# Autodesk Inventor assembly: Neuronexus
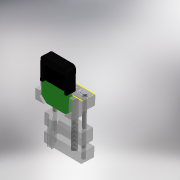
[picture p0: Inventor's stored thumbnail of the model, 180x180]
Saved by Autodesk Inventor 2020 (Build 240168000, 168)
## iProperties
Created: 2020-02-24
Part Number: Neuronexus
Document SubType Name: Assembly
Designer: Knowblesse
Author: Knowblesse
## Documents named in this file (7)
- C:\VCF\Microdrive\Neuronexus\Neuronexus.iam
- C:\VCF\Microdrive\Neuronexus\Bot.ipt
- C:\VCF\Microdrive\Neuronexus\Mid.ipt
- C:\VCF\Microdrive\Neuronexus\Screw.ipt
- C:\VCF\Microdrive\Neuronexus\Top.ipt
- C:\VCF\Microdrive\Neuronexus\19G_Pillar.ipt
- C:\VCF\Microdrive\Neuronexus\Probe.ipt
## Components (7 placed, 6 different names)
1. Bot:1 — 회전:4, 회전:5
2. Mid:1 — 원통형:2, 원통형:3
3. Screw:1 — 회전:1
4. Top:1 — 회전:1, 메이트:1, 회전:2, 회전:3, 강체:1
5. 19G_Pillar:1 — 메이트:1, 회전:3, 회전:4, 원통형:3
6. 19G_Pillar:2 — 원통형:2, 회전:2, 회전:5
7. Probe:1 — 강체:1
## Relationships (9: RevoluteJoint 5, CylindricalJoint 2, Mate 1, WeldJoint 1)
- 원통형:2 [CylindricalJoint]: Mid:1 ↔ 19G_Pillar:2
- 회전:1 [RevoluteJoint]: Screw:1 ↔ Top:1
- 메이트:1 [Mate]: Top:1 ↔ 19G_Pillar:1
- 회전:2 [RevoluteJoint]: Top:1 ↔ 19G_Pillar:2
- 회전:3 [RevoluteJoint]: Top:1 ↔ 19G_Pillar:1
- 회전:4 [RevoluteJoint]: Bot:1 ↔ 19G_Pillar:1
- 회전:5 [RevoluteJoint]: Bot:1 ↔ 19G_Pillar:2
- 원통형:3 [CylindricalJoint]: Mid:1 ↔ 19G_Pillar:1
- 강체:1 [WeldJoint]: Top:1 ↔ Probe:1
